# Autodesk Inventor assembly: board_outline
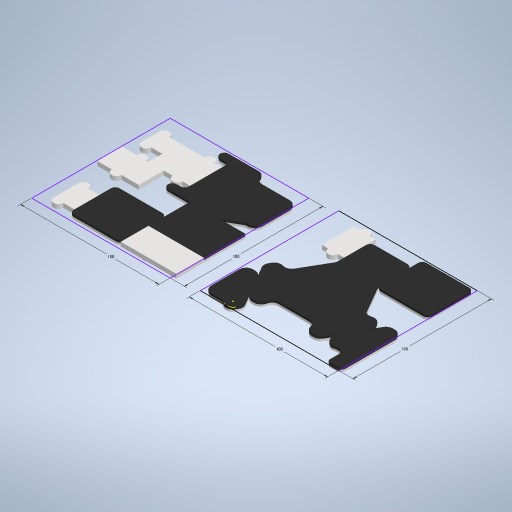
[picture p0: Inventor's stored thumbnail of the model, 512x512]
Saved by Autodesk Inventor 2024.1 (Build 281209000, 209)
## iProperties
Created: 2025-04-11
Part Number: board_outline
Document SubType Name: Assembly
Designer: hibik
Author: hibik
## Documents named in this file (14)
- C:\Users\hibik\Documents\Robomech\RESCUE\ORCA\hard\board\CORE\board_outline.iam
- C:\Users\hibik\Documents\Robomech\RESCUE\ORCA\hard\board\CORE\CORE_outline.ipt
- C:\Users\hibik\Documents\Robomech\RESCUE\ORCA\hard\board\CORE\CORE_hat_outline.ipt
- C:\Users\hibik\Documents\Robomech\RESCUE\ORCA\hard\board\CORE\CORE_hat_right.ipt
- C:\Users\hibik\Documents\Robomech\RESCUE\ORCA\hard\board\CORE\CORE_hat_upper_outline.ipt
- C:\Users\hibik\Documents\Robomech\RESCUE\ORCA\hard\board\CORE\CORE_md.ipt
- C:\Users\hibik\Documents\Robomech\RESCUE\ORCA\hard\board\CORE\CORE_arm.ipt
- C:\Users\hibik\Documents\Robomech\RESCUE\ORCA\hard\board\CORE\CORE_set_outline.ipt
- C:\Users\hibik\Documents\Robomech\RESCUE\ORCA\hard\board\CORE\external_input.ipt
- C:\Users\hibik\Documents\Robomech\RESCUE\ORCA\hard\board\CORE\led.ipt
- C:\Users\hibik\Documents\Robomech\RESCUE\ORCA\hard\board\CORE\reset.ipt
- C:\Users\hibik\Documents\Robomech\RESCUE\ORCA\hard\board\CORE\type_A.ipt
- C:\Users\hibik\Documents\Robomech\RESCUE\ORCA\hard\board\CORE\type_C.ipt
- C:\Users\hibik\Documents\Robomech\RESCUE\ORCA\hard\board\CORE\voltage_hub.ipt
## Components (14 placed, 13 different names)
1. CORE_outline:1 — フラッシュ:1, フラッシュ:2, メイト:1, メイト:2, 正接:3, フラッシュ:13, フラッシュ:14, フラッシュ:15, フラッシュ:16, メイト:11, メイト:13
2. CORE_hat_outline:1 — フラッシュ:1, メイト:1, 正接:3, メイト:10, フラッシュ:26
3. CORE_hat_right:1 — フラッシュ:2, メイト:2, メイト:10, メイト:22, メイト:23
4. CORE_set_outline:1 — フラッシュ:9, フラッシュ:10, フラッシュ:11
5. external_input:1 — フラッシュ:16, メイト:13, 正接:4
6. reset:1 — メイト:20, 正接:6
7. voltage_hub:1 — フラッシュ:18, メイト:17, メイト:18, フラッシュ:23, フラッシュ:26, メイト:22
8. CORE_md:4 — フラッシュ:14, メイト:11, 正接:4, メイト:23
9. CORE_md:5 — フラッシュ:15, メイト:18, メイト:19, フラッシュ:23, メイト:20, 正接:6
10. CORE_arm:2 — フラッシュ:13, フラッシュ:18, メイト:17, メイト:19, フラッシュ:27, メイト:25, フラッシュ:28, メイト:29
11. CORE_hat_upper_outline:3 — フラッシュ:27, メイト:25, フラッシュ:28, フラッシュ:29, フラッシュ:30, メイト:26, フラッシュ:33
12. type_A:2 — フラッシュ:30, メイト:26, メイト:27, フラッシュ:32, フラッシュ:33, メイト:28
13. led:2 — フラッシュ:31, メイト:27, フラッシュ:32
14. type_C:2 — フラッシュ:29, フラッシュ:31, メイト:28, メイト:29
## Relationships (38: Flush 19, Mate 16, Tangent 3)
- フラッシュ:1 [Flush]: CORE_outline:1 ↔ CORE_hat_outline:1
- フラッシュ:2 [Flush]: CORE_outline:1 ↔ CORE_hat_right:1
- メイト:1 [Mate]: CORE_outline:1 ↔ CORE_hat_outline:1
- メイト:2 [Mate]: CORE_outline:1 ↔ CORE_hat_right:1
- 正接:3 [Tangent]: CORE_outline:1 ↔ CORE_hat_outline:1
- フラッシュ:9 [Flush]: CORE_set_outline:1
- フラッシュ:10 [Flush]: CORE_set_outline:1
- フラッシュ:11 [Flush]: CORE_set_outline:1
- メイト:10 [Mate] (-99 mm): CORE_hat_outline:1 ↔ CORE_hat_right:1
- フラッシュ:13 [Flush]: CORE_outline:1 ↔ CORE_arm:2
- フラッシュ:14 [Flush]: CORE_outline:1 ↔ CORE_md:4
- フラッシュ:15 [Flush]: CORE_outline:1 ↔ CORE_md:5
- フラッシュ:16 [Flush]: CORE_outline:1 ↔ external_input:1
- メイト:11 [Mate]: CORE_outline:1 ↔ CORE_md:4
- メイト:13 [Mate]: CORE_outline:1 ↔ external_input:1
- 正接:4 [Tangent]: external_input:1 ↔ CORE_md:4
- フラッシュ:18 [Flush]: voltage_hub:1 ↔ CORE_arm:2
- メイト:17 [Mate]: voltage_hub:1 ↔ CORE_arm:2
- メイト:18 [Mate]: voltage_hub:1 ↔ CORE_md:5
- メイト:19 [Mate]: CORE_md:5 ↔ CORE_arm:2
- フラッシュ:23 [Flush]: voltage_hub:1 ↔ CORE_md:5
- メイト:20 [Mate]: reset:1 ↔ CORE_md:5
- フラッシュ:26 [Flush]: CORE_hat_outline:1 ↔ voltage_hub:1
- メイト:22 [Mate] (20 mm): CORE_hat_right:1 ↔ voltage_hub:1
- 正接:6 [Tangent]: reset:1 ↔ CORE_md:5
- メイト:23 [Mate] (-94 mm): CORE_hat_right:1 ↔ CORE_md:4
- フラッシュ:27 [Flush]: CORE_arm:2 ↔ CORE_hat_upper_outline:3
- メイト:25 [Mate]: CORE_arm:2 ↔ CORE_hat_upper_outline:3
- フラッシュ:28 [Flush]: CORE_arm:2 ↔ CORE_hat_upper_outline:3
- フラッシュ:29 [Flush]: CORE_hat_upper_outline:3 ↔ type_C:2
- フラッシュ:30 [Flush]: CORE_hat_upper_outline:3 ↔ type_A:2
- フラッシュ:31 [Flush]: led:2 ↔ type_C:2
- メイト:26 [Mate]: CORE_hat_upper_outline:3 ↔ type_A:2
- メイト:27 [Mate]: type_A:2 ↔ led:2
- フラッシュ:32 [Flush]: type_A:2 ↔ led:2
- フラッシュ:33 [Flush] (11 mm): CORE_hat_upper_outline:3 ↔ type_A:2
- メイト:28 [Mate]: type_A:2 ↔ type_C:2
- メイト:29 [Mate] (-99 mm): CORE_arm:2 ↔ type_C:2
